# Autodesk Inventor assembly: X-belt tensioner
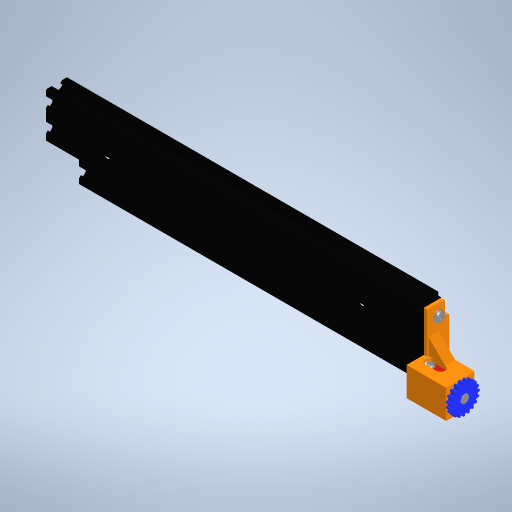
[picture p0: Inventor's stored thumbnail of the model, 512x512]
Saved by Autodesk Inventor 2023 (Build 270158000, 158)
## iProperties
Created: 2023-03-07
Part Number: X-belt tensioner
Document SubType Name: Assembly
Designer: Josh
Author: Josh
## Documents named in this file (9)
- C:\Users\Josh\Documents\Inventor\Mingda\X-belt tensioner.iam
- C:\Users\Josh\Documents\Inventor\Mingda\X_belt1.ipt
- C:\Users\Josh\Documents\Inventor\Mingda\20x60x342.ipt
- C:\Users\Josh\Documents\Inventor\Mingda\X_belt2.ipt
- C:\Users\Josh\Documents\Inventor\Mingda\Pulley.ipt
- C:\Users\Josh\Documents\Inventor\Content Center Files\R2023\ru-RU\ANSI B18.3.4M(1)\ANSI B18.3.4M - M4 x 0.7 x 20(2).ipt
- C:\Users\Josh\Documents\Inventor\Content Center Files\R2023\ru-RU\ANSI B18.3.4M(1)\ANSI B18.3.4M - M5 x 0.8 x 8(2).ipt
- C:\Users\Josh\Documents\Inventor\Content Center Files\R2023\ru-RU\ANSI B 18.2.4.1 M(1)\ANSI B 18.2.4.1 M - M4 x 0.7Style 1.ipt
- C:\Users\Josh\Documents\Inventor\Mingda\X_belt3.ipt
## Components (10 placed, 8 different names)
1. X_belt1:1 — Совмещение:1, Совмещение:2, Совмещение:3, Совмещение:6, Угол:1, Вставка:3, Вставка:4, Совмещение:10
2. 20x60x342:1 — Совмещение:1, Совмещение:2, Совмещение:3, Совмещение:7, Заподлицо:1, Заподлицо:2, Совмещение:8
3. X_belt2:1 — Совмещение:4, Совмещение:5, Совмещение:6, Угол:1, Совмещение:8, Вставка:1, Вставка:2, 1
4. Pulley:1 — Совмещение:4, Совмещение:5
5. M4 x 0.7 x 20:1 — Вставка:1
6. M4 x 0.7 x 20:2 — Вставка:2, Совмещение:9, Совмещение:12
7. M5 x 0.8 x 8:1 — Вставка:3
8. M4 x 0.7 x 20:3 — Вставка:4
9. Hex nut M4 x 0.7:1 — 1, Угол:2, Совмещение:11, Совмещение:12
10. X_belt3:1 — Совмещение:9, Совмещение:10, Угол:2, Совмещение:11
## Relationships (21: Mate 12, Insert 4, Flush 2, Angle 2, RelateRotateTranslate 1)
- Совмещение:1 [Mate]: X_belt1:1 ↔ 20x60x342:1
- Совмещение:2 [Mate]: X_belt1:1 ↔ 20x60x342:1
- Совмещение:3 [Mate]: X_belt1:1 ↔ 20x60x342:1
- Совмещение:4 [Mate]: X_belt2:1 ↔ Pulley:1
- Совмещение:5 [Mate] (0.425 mm): X_belt2:1 ↔ Pulley:1
- Совмещение:6 [Mate]: X_belt1:1 ↔ X_belt2:1
- Совмещение:7 [Mate]: 20x60x342:1
- Заподлицо:1 [Flush]: 20x60x342:1
- Угол:1 [Angle] (0 deg): X_belt1:1 ↔ X_belt2:1
- Заподлицо:2 [Flush]: 20x60x342:1
- Совмещение:8 [Mate]: 20x60x342:1 ↔ X_belt2:1
- Вставка:1 [Insert]: X_belt2:1 ↔ M4 x 0.7 x 20:1
- Вставка:2 [Insert]: X_belt2:1 ↔ M4 x 0.7 x 20:2
- Вставка:3 [Insert]: X_belt1:1 ↔ M5 x 0.8 x 8:1
- Вставка:4 [Insert]: X_belt1:1 ↔ M4 x 0.7 x 20:3
- 1 [RelateRotateTranslate] (10.185 mm): X_belt2:1 ↔ Hex nut M4 x 0.7:1
- Совмещение:9 [Mate]: M4 x 0.7 x 20:2 ↔ X_belt3:1
- Совмещение:10 [Mate]: X_belt1:1 ↔ X_belt3:1
- Угол:2 [Angle] (0 deg): Hex nut M4 x 0.7:1 ↔ X_belt3:1
- Совмещение:11 [Mate]: Hex nut M4 x 0.7:1 ↔ X_belt3:1
- Совмещение:12 [Mate]: M4 x 0.7 x 20:2 ↔ Hex nut M4 x 0.7:1
